# Autodesk Inventor assembly: RCU
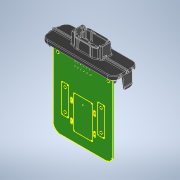
[picture p0: Inventor's stored thumbnail of the model, 180x180]
Saved by Autodesk Inventor 2021 (Build 250183000, 183)
## iProperties
Created: 2020-09-13
Part Number: RCU
Document SubType Name: Assembly
Designer: Viktor
Author: Viktor
## Documents named in this file (6)
- C:\Users\Viktor\Documents\GitHub\WaveRunner-CCU\RCU\hw\CAD\RCU.iam
- C:\Users\Viktor\Documents\GitHub\WaveRunner-CCU\RCU\hw\CAD\c-eec-325x4a-e016-99-3d.ipt
- C:\Users\Viktor\Documents\GitHub\WaveRunner-CCU\RCU\hw\CAD\FrSky_RX8R.ipt
- C:\Users\Viktor\Documents\GitHub\WaveRunner-CCU\RCU\hw\CAD\PCB.ipt
- C:\Users\Viktor\Documents\GitHub\WaveRunner-CCU\RCU\hw\CAD\c-dtm13-12pa-r008-c-3d.ipt
- C:\Users\Viktor\Documents\GitHub\WaveRunner-CCU\RCU\hw\CAD\AntennaHolder.ipt
## Components (6 placed, 5 different names)
1. c-eec-325x4a-e016-99-3d:1 — Rigid:2
2. FrSky_RX8R:1 — Mate:1, Mate:2, Mate:3
3. PCB:1 — Rigid:1, Rigid:3, Rigid:4, Mate:1, Mate:2, Mate:3
4. c-dtm13-12pa-r008-c-3d:2 — Rigid:1, Rigid:2
5. AntennaHolder:1 — Rigid:3
6. AntennaHolder:2 — Rigid:4
## Relationships (7: WeldJoint 4, Mate 3)
- Rigid:1 [WeldJoint] (-0.381 mm): PCB:1 ↔ c-dtm13-12pa-r008-c-3d:2
- Rigid:2 [WeldJoint]: c-eec-325x4a-e016-99-3d:1 ↔ c-dtm13-12pa-r008-c-3d:2
- Rigid:3 [WeldJoint]: PCB:1 ↔ AntennaHolder:1
- Rigid:4 [WeldJoint]: PCB:1 ↔ AntennaHolder:2
- Mate:1: FrSky_RX8R:1 ↔ PCB:1
- Mate:2: FrSky_RX8R:1 ↔ PCB:1
- Mate:3: FrSky_RX8R:1 ↔ PCB:1
